# Autodesk Inventor assembly: Assembly1
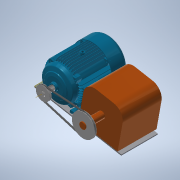
[picture p0: Inventor's stored thumbnail of the model, 180x180]
Saved by Autodesk Inventor 2020 (Build 240168000, 168)
## iProperties
Created: 2017-11-11
Part Number: Assembly1
Document SubType Name: Assembly
Designer: Mr.Duc
Author: Mr.Duc
## Documents named in this file (13)
- C:\Users\DanielAlvaradoPelaez\Desktop\Espol S5\diseño y simulacion de maquinas\deber\tarea 4\ac-motor-14.snapshot.1\Assembly1.iam
- C:\Users\DanielAlvaradoPelaez\Desktop\Espol S5\diseño y simulacion de maquinas\deber\tarea 4\ac-motor-14.snapshot.1\nap sau.ipt
- C:\Users\DanielAlvaradoPelaez\Desktop\Espol S5\diseño y simulacion de maquinas\deber\tarea 4\ac-motor-14.snapshot.1\than.ipt
- C:\Users\Mr.Duc\Documents\Inventor\Content Center Files\R2018\en-US\ISO 7046-1(1)\DIN EN ISO 7046-1 - M8 x 14 - 4.8 - H.ipt
- E:\Inventor 2017\VHD INVENTOR\DACTM\DONG CO\Assembly1\Design Accelerator\Bearing1.iam
- C:\Users\DanielAlvaradoPelaez\Desktop\Espol S5\diseño y simulacion de maquinas\deber\tarea 4\ac-motor-14.snapshot.1\truc.ipt
- C:\Users\DanielAlvaradoPelaez\Desktop\Espol S5\diseño y simulacion de maquinas\deber\tarea 4\ac-motor-14.snapshot.1\nap truoc.ipt
- C:\Users\Mr.Duc\Documents\Inventor\Content Center Files\R2018\en-US\BS EN ISO 4016\BS EN ISO 4016 - M10x65.ipt
- C:\Users\Mr.Duc\Documents\Inventor\Content Center Files\R2018\en-US\ISO 4032(2)\ISO 4032 - M10 - ISO.ipt
- E:\Inventor 2017\VHD INVENTOR\DACTM\DONG CO\long soc.ipt
- C:\Users\DanielAlvaradoPelaez\Desktop\Espol S5\diseño y simulacion de maquinas\deber\tarea 4\ac-motor-14.snapshot.1\Pieza2.ipt
- C:\Users\DanielAlvaradoPelaez\Desktop\Espol S5\diseño y simulacion de maquinas\deber\tarea 4\ac-motor-14.snapshot.1\Pieza3.ipt
- C:\Users\DanielAlvaradoPelaez\Desktop\Espol S5\diseño y simulacion de maquinas\deber\tarea 4\ac-motor-14.snapshot.1\Assembly1\Design Accelerator\Transmisión de correa trapezoidal1.iam
## Components (21 placed, 12 different names)
1. nap sau:1 — Mate:1, Mate:2, Mate:3, Mate:4, Mate:6, Mate:7
2. than:1 — Mate:1, Mate:2, Mate:8, Mate:9, Mate:10, Mate:11, Mate:12, Flush:2, Mate:14, Mate:16, Mate:17, Mate:18, Insert:2, Flush:3, Nivelación:6, Nivelación:7, Nivelación:8, Nivelación:9
3. DIN EN ISO 7046-1 H M8 x 14 - 4.8 - H:4 — Mate:3, Mate:10
4. DIN EN ISO 7046-1 H M8 x 14 - 4.8 - H:2 — Mate:4, Mate:9
5. DIN EN ISO 7046-1 H M8 x 14 - 4.8 - H:3 — Mate:6, Mate:11
6. DIN EN ISO 7046-1 H M8 x 14 - 4.8 - H:1 — Mate:7, Mate:8
7. Bearing:1 [sub-assembly] — Mate:12, Flush:2, Mate:13
8. truc:1 — Mate:13, Mate:14, Mate:15, Coincidencia:19
9. nap truoc:1 — Mate:15, Mate:16, Mate:17, Mate:18, Insert:1
10. long soc:1 — Flush:3
11. Pieza2:1 — Nivelación:6, Nivelación:7, Nivelación:8, Nivelación:9, Nivelación:10, Nivelación:12, Nivelación:13
12. Pieza3:1 — Nivelación:11, Nivelación:12, Nivelación:13, Coincidencia:19
13. Transmisión de correa trapezoidal:1 [sub-assembly]
14. BS EN ISO 4016 M10x65:1 — Insert:1
15. BS EN ISO 4016 M10x65:2
16. BS EN ISO 4016 M10x65:3
17. BS EN ISO 4016 M10x65:4
18. ISO 4032 M10:1 — Insert:2
19. ISO 4032 M10:2
20. ISO 4032 M10:3
21. ISO 4032 M10:4
## Component patterns: (4 elements, first: BS EN ISO 4016 M10x65:1), (4 elements, first: ISO 4032 M10:1)
## Relationships (30: Mate 18, Flush 10, Insert 2)
- Mate:1: nap sau:1 ↔ than:1
- Mate:2: nap sau:1 ↔ than:1
- Mate:3: nap sau:1 ↔ DIN EN ISO 7046-1 H M8 x 14 - 4.8 - H:4
- Mate:4: nap sau:1 ↔ DIN EN ISO 7046-1 H M8 x 14 - 4.8 - H:2
- Mate:6: nap sau:1 ↔ DIN EN ISO 7046-1 H M8 x 14 - 4.8 - H:3
- Mate:7: nap sau:1 ↔ DIN EN ISO 7046-1 H M8 x 14 - 4.8 - H:1
- Mate:8 (0.5 mm): than:1 ↔ DIN EN ISO 7046-1 H M8 x 14 - 4.8 - H:1
- Mate:9 (0.5 mm): than:1 ↔ DIN EN ISO 7046-1 H M8 x 14 - 4.8 - H:2
- Mate:10 (0.5 mm): than:1 ↔ DIN EN ISO 7046-1 H M8 x 14 - 4.8 - H:4
- Mate:11 (0.5 mm): than:1 ↔ DIN EN ISO 7046-1 H M8 x 14 - 4.8 - H:3
- Mate:12: than:1 ↔ Bearing:1
- Flush:2: than:1 ↔ Bearing:1
- Mate:13: Bearing:1 ↔ truc:1
- Mate:14: than:1 ↔ truc:1
- Mate:15: truc:1 ↔ nap truoc:1
- Mate:16: than:1 ↔ nap truoc:1
- Mate:17: than:1 ↔ nap truoc:1
- Mate:18: than:1 ↔ nap truoc:1
- Insert:1: nap truoc:1 ↔ BS EN ISO 4016 M10x65:1
- Insert:2: than:1 ↔ ISO 4032 M10:1
- Flush:3: than:1 ↔ long soc:1
- Nivelación:6 [Flush]: than:1 ↔ Pieza2:1
- Nivelación:7 [Flush]: than:1 ↔ Pieza2:1
- Nivelación:8 [Flush] (10 mm): than:1 ↔ Pieza2:1
- Nivelación:9 [Flush] (30 mm): than:1 ↔ Pieza2:1
- Nivelación:10 [Flush] (187.965 mm): Pieza2:1
- Nivelación:11 [Flush]: Pieza3:1
- Nivelación:12 [Flush]: Pieza2:1 ↔ Pieza3:1
- Nivelación:13 [Flush]: Pieza2:1 ↔ Pieza3:1
- Coincidencia:19 [Mate] (373 mm): truc:1 ↔ Pieza3:1
